# Autodesk Inventor assembly: MG-Akku 6S1P Tattu Funfly 1550mAh
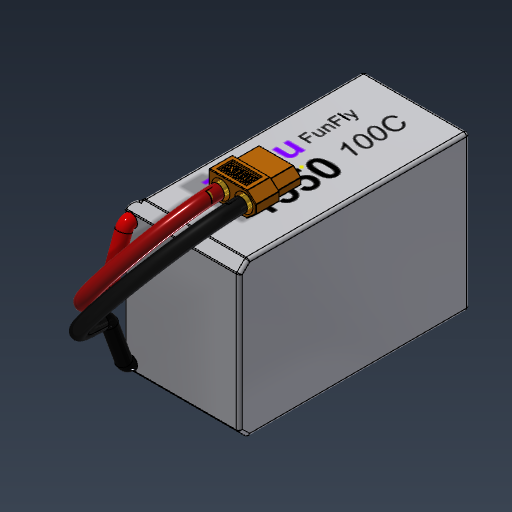
[picture p0: Inventor's stored thumbnail of the model, 512x512]
Saved by Autodesk Inventor 2023.1 (Build 271208000, 208)
## iProperties
Part Number: MG-Akku 6S1P Tattu Funfly 1550mAh
Material: Generisch
Document SubType Name: Assembly
Designer: rYan
Mass: 251.621 g
Surface Area: 167.344 cm^2
Volume: 116.033 cm^3
Density: 2.16853 g/cm^3
Author: rYan
## Documents named in this file (4)
- D:\TIGERsGIT\Hardware\mechanik\2020\Inventor\Purchased Parts\MG-Akku 6S1P Tattu Funfly 1550mAh.iam
- D:\TIGERsGIT\Hardware\mechanik\2020\Inventor\Purchased Parts\XT60 Buchse.ipt
- D:\TIGERsGIT\Hardware\mechanik\2020\Inventor\Purchased Parts\Akku 6S1P Tattu Funfly 1550mAh.ipt
- D:\TIGERsGIT\Hardware\mechanik\2020\Inventor\Purchased Parts\MG-Akku 6S1P Tattu Funfly 1550mAh\AIP\Kabel und Kabelbaum\MG-Akku 6S1P Tattu Funfly 1550mAh.Kabelbaum.iam
## Components (3 placed, 3 different names)
1. Akku 6S1P Tattu Funfly 1550mAh:2 — Fluchtend:1, Fluchtend:2, Fluchtend:3
2. XT60 Buchse:1
3. MG-Akku 6S1P Tattu Funfly 1550mAh.Kabelbaum [sub-assembly]
## Relationships (5: Flush 3, Mate 2)
- [Mate] (2 mm): Akku 6S1P Tattu Funfly 1550mAh:2 ↔ XT60 Buchse:1
- [Mate] (-5 mm): Akku 6S1P Tattu Funfly 1550mAh:2 ↔ XT60 Buchse:1
- Fluchtend:1 [Flush]: Akku 6S1P Tattu Funfly 1550mAh:2
- Fluchtend:2 [Flush]: Akku 6S1P Tattu Funfly 1550mAh:2
- Fluchtend:3 [Flush]: Akku 6S1P Tattu Funfly 1550mAh:2
